# Autodesk Inventor assembly: motor wheel assembly2
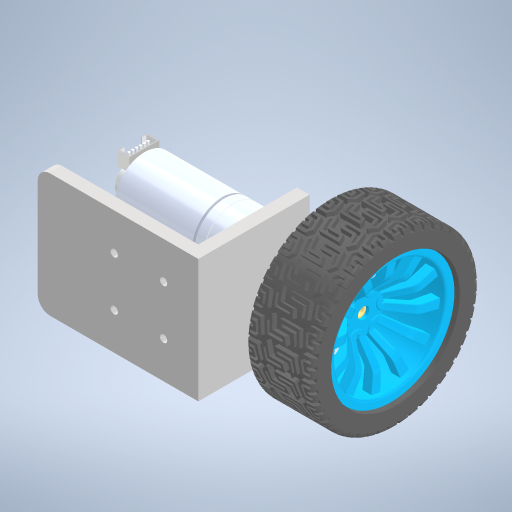
[picture p0: Inventor's stored thumbnail of the model, 512x512]
Saved by Autodesk Inventor 2023.2 (Build 272271000, 271)
## iProperties
Created: 2024-08-13
Part Number: motor wheel assembly2
Document SubType Name: Assembly
Designer: PC
Author: PC
## Documents named in this file (5)
- C:\Users\PC\Desktop\motor wheel assembly2.iam
- C:\Users\PC\Desktop\65mm蓝色轮胎总装-实际外径68mm.iam
- C:\Users\PC\Desktop\motor wheel connector.ipt
- C:\Users\PC\Desktop\Motor.ipt
- C:\Users\PC\Desktop\motor chassis holder1.ipt
## Components (4 placed, 4 different names)
1. 65mm蓝色轮胎总装-实际外径68mm:1 [sub-assembly] — Insert:1
2. motor wheel connector:1 — Insert:1, Insert:2
3. Motor:1 — Insert:2, Insert:3
4. motor chassis holder1:1 — Insert:3
## Relationships (3: Insert 3)
- Insert:1 (-12 mm): 65mm蓝色轮胎总装-实际外径68mm:1 ↔ motor wheel connector:1
- Insert:2 (-10 mm): motor wheel connector:1 ↔ Motor:1
- Insert:3 (-2.7 mm): Motor:1 ↔ motor chassis holder1:1
